# Autodesk Inventor assembly: Custom Cover Assembly
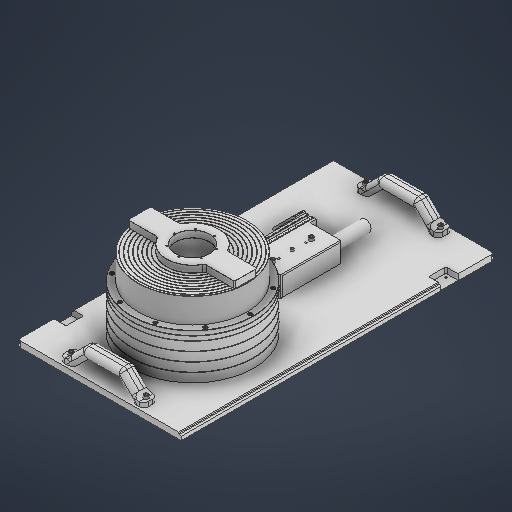
[picture p0: Inventor's stored thumbnail of the model, 512x512]
Saved by Autodesk Inventor 2025 (Build 290162000, 162)
## iProperties
Created: 2024-04-26
Part Number: Custom Cover Assembly
Document SubType Name: Assembly
Designer: Thienan Hoang
Author: Thienan Hoang
## Documents named in this file (23)
- C:\Users\mayhe\OneDrive\Documents\GitHub\In-situ-monitoring-of-powder-bed-fusion-additive-manufacturing\system_development\custom-cover\v0.1\hardware design\Custom Cover Full Assembly.iam
- C:\Users\mayhe\OneDrive\Documents\GitHub\In-situ-monitoring-of-powder-bed-fusion-additive-manufacturing\system_development\custom-cover\v0.1\hardware design\cover\Updated Cover.ipt
- C:\Users\mayhe\OneDrive\Documents\GitHub\In-situ-monitoring-of-powder-bed-fusion-additive-manufacturing\system_development\laser-vibrometer\v0.1\Hardware_design\Updated Laser Scanner.ipt
- C:\Users\mayhe\OneDrive\Documents\GitHub\In-situ-monitoring-of-powder-bed-fusion-additive-manufacturing\system_development\laser-vibrometer\v0.1\Hardware_design\Updated Laser Bracket.ipt
- C:\Users\mayhe\OneDrive\Documents\GitHub\In-situ-monitoring-of-powder-bed-fusion-additive-manufacturing\system_development\custom-cover\v0.1\hardware design\fasteners-standoffs\25-4136.ipt
- C:\Users\mayhe\OneDrive\Documents\GitHub\In-situ-monitoring-of-powder-bed-fusion-additive-manufacturing\system_development\custom-cover\v0.1\hardware design\fasteners-standoffs\11-4310.ipt
- C:\Users\mayhe\OneDrive\Documents\GitHub\In-situ-monitoring-of-powder-bed-fusion-additive-manufacturing\system_development\custom-cover\v0.1\hardware design\8020-parts\20-2020-160-CL.ipt
- C:\Users\mayhe\OneDrive\Documents\GitHub\In-situ-monitoring-of-powder-bed-fusion-additive-manufacturing\system_development\custom-cover\v0.1\hardware design\8020-parts\14159_m.ipt
- C:\Users\mayhe\OneDrive\Documents\GitHub\In-situ-monitoring-of-powder-bed-fusion-additive-manufacturing\system_development\galvo-scanner\V0.1\hardware design\GVS102.iam
- C:\Users\mayhe\OneDrive\Documents\GitHub\In-situ-monitoring-of-powder-bed-fusion-additive-manufacturing\system_development\custom-cover\v0.1\hardware design\8020-parts\20-2020-200-CL.ipt
- C:\Users\mayhe\OneDrive\Documents\GitHub\In-situ-monitoring-of-powder-bed-fusion-additive-manufacturing\system_development\custom-cover\v0.1\hardware design\8020-parts\25-1964.ipt
- C:\Users\mayhe\OneDrive\Documents\GitHub\In-situ-monitoring-of-powder-bed-fusion-additive-manufacturing\system_development\custom-cover\v0.1\hardware design\cylinder-parts\whole-pieces\Cylinder Spacer Bottom.ipt
- C:\Users\mayhe\OneDrive\Documents\GitHub\In-situ-monitoring-of-powder-bed-fusion-additive-manufacturing\system_development\custom-cover\v0.1\hardware design\cylinder-parts\whole-pieces\Cylinder Spacer Top.ipt
- C:\Users\mayhe\OneDrive\Documents\GitHub\In-situ-monitoring-of-powder-bed-fusion-additive-manufacturing\system_development\custom-cover\v0.1\hardware design\cylinder-parts\whole-pieces\Cylinder Slidey Bit.iam
- C:\Users\mayhe\OneDrive\Documents\GitHub\In-situ-monitoring-of-powder-bed-fusion-additive-manufacturing\system_development\custom-cover\v0.1\hardware design\cylinder-parts\whole-pieces\Cylinder Spacer 25mm.ipt
- C:\Users\mayhe\OneDrive\Documents\GitHub\In-situ-monitoring-of-powder-bed-fusion-additive-manufacturing\system_development\custom-cover\v0.1\hardware design\cylinder-parts\whole-pieces\Head Thing.ipt
- C:\Users\mayhe\OneDrive\Documents\GitHub\In-situ-monitoring-of-powder-bed-fusion-additive-manufacturing\system_development\custom-cover\v0.1\hardware design\cylinder-parts\whole-pieces\Cylinder Bottom.ipt
- C:\Users\mayhe\OneDrive\Documents\GitHub\In-situ-monitoring-of-powder-bed-fusion-additive-manufacturing\system_development\custom-cover\v0.1\hardware design\cover\Handles.ipt
- C:\Users\mayhe\OneDrive\Documents\GitHub\In-situ-monitoring-of-powder-bed-fusion-additive-manufacturing\system_development\custom-cover\v0.1\hardware design\fasteners-standoffs\ANSI B18.3.1M - M2x0.4 x 20(1).ipt
- C:\Users\mayhe\OneDrive\Documents\GitHub\In-situ-monitoring-of-powder-bed-fusion-additive-manufacturing\system_development\custom-cover\v0.1\hardware design\fasteners-standoffs\ANSI B18.3.1M - M6x1 x 20(1).ipt
- C:\Users\mayhe\OneDrive\Documents\GitHub\In-situ-monitoring-of-powder-bed-fusion-additive-manufacturing\system_development\custom-cover\v0.1\hardware design\fasteners-standoffs\ANSI B18.3.1M - M6x1 x 10(1).ipt
- C:\Users\mayhe\OneDrive\Documents\GitHub\In-situ-monitoring-of-powder-bed-fusion-additive-manufacturing\system_development\custom-cover\v0.1\hardware design\fasteners-standoffs\ANSI B18.3.1M - M4x0.7 x 6(1).ipt
- C:\Users\mayhe\OneDrive\Documents\GitHub\In-situ-monitoring-of-powder-bed-fusion-additive-manufacturing\system_development\custom-cover\v0.1\hardware design\fasteners-standoffs\ANSI B18.3.1M - M5x0.8 x 100(1).ipt
## Components (58 placed, 22 different names)
1. Updated Cover:1 — Mate:15, Mate:17, Mate:18, Mate:19, Mate:20, Mate:32, Mate:33, Flush:5, Mate:48, Mate:82, Mate:86, Mate:98, Mate:106, Mate:107, Mate:108, Mate:109
2. 11-4310:10 — Mate:125
3. 11-4310:11 — Mate:126
4. 11-4310:12 — Mate:127
5. 11-4310:13 — Mate:128
6. GVS102:1 [sub-assembly] — Mate:66, Mate:67, Angle:2
7. 20-2020-200-CL:1 — Mate:69, Flush:8, Mate:85, Angle:2, Mate:122, Mate:123, Mate:124
8. 25-1964:1 — Mate:66, Mate:67, Mate:69, Flush:8, Mate:85
9. Updated Laser Bracket:1 — Flush:9, Mate:83, Rotational:15, Mate:86, Insert:22, Insert:23, Insert:24, Mate:125, Mate:126, Mate:127, Mate:128
10. Updated Laser Scanner:1 — Rotational:15
11. Head Thing:1 — Mate:110, Mate:111, Insert:11, Insert:12, Insert:13, Insert:14, Insert:15, Insert:16, Insert:17
12. Cylinder Bottom:1 — Mate:98, Mate:99, Mate:100
13. Cylinder Spacer Bottom:1 — Mate:99, Mate:100, Mate:101, Mate:102, Mate:122, Mate:123, Mate:124
14. Cylinder Spacer Top:1 — Mate:101, Mate:102, Mate:103, Mate:104
15. Cylinder Spacer 25mm:1 — Mate:103, Mate:104, Mate:105, Rotational:16
16. Cylinder Slidey Bit:1 [sub-assembly] — Mate:105, Rotational:16, Mate:110, Mate:111, Mate:112, Mate:113, Mate:114, Mate:115, Mate:116, Mate:117, Mate:118, Mate:119, Mate:120, Mate:121
17. Handles:1 — Mate:108, Mate:109, Insert:18, Insert:19
18. Handles:2 — Mate:106, Mate:107, Insert:20, Insert:21
19. 25-4136:1 — Mate:5, Mate:6, Mate:9, Mate:10, Flush:1, Flush:2, Mate:15, Mate:17, Mate:18, Rotational:2, Rigid:1
20. 20-2020-160-CL:1 — Flush:1, Mate:11, Mate:12, Flush:9, Mate:83
21. 11-4310:1 — Mate:5, Mate:8
22. 11-4310:2 — Mate:6, Mate:7
23. 14159_m:1 — Mate:8, Mate:10, Mate:13, Mate:14
24. 14159_m:2 — Mate:7, Mate:9, Mate:11, Mate:12
25. 20-2020-160-CL:2 — Flush:2, Mate:13, Mate:14, Mate:56
26. 11-4310:3 — Rotational:2
27. 11-4310:4 — Rigid:1
28. 25-4136:3 — Mate:19, Mate:20, Rotational:3, Rotational:4, Rotational:5, Rotational:6, Mate:23, Mate:32, Mate:33, Mate:82
29. 11-4310:6 — Rotational:3
30. 11-4310:7 — Rotational:4
31. 11-4310:8 — Rotational:5, Mate:21
32. 11-4310:9 — Rotational:6, Mate:22
33. 14159_m:3 — Mate:22, Mate:56
34. 14159_m:4 — Mate:21, Mate:23
35. Forged Socket Head Cap Screw - Metric M2x0.4 x 20:1 — Insert:11
36. Forged Socket Head Cap Screw - Metric M2x0.4 x 20:2 — Insert:12
37. Forged Socket Head Cap Screw - Metric M2x0.4 x 20:3 — Insert:13
38. Forged Socket Head Cap Screw - Metric M2x0.4 x 20:4 — Insert:14
39. Forged Socket Head Cap Screw - Metric M2x0.4 x 20:5 — Insert:15
40. Forged Socket Head Cap Screw - Metric M2x0.4 x 20:6 — Insert:16
41. Forged Socket Head Cap Screw - Metric M2x0.4 x 20:7 — Insert:17
42. Forged Socket Head Cap Screw - Metric M6x1 x 20:1 — Insert:18
43. Forged Socket Head Cap Screw - Metric M6x1 x 20:2 — Insert:19
44. Forged Socket Head Cap Screw - Metric M6x1 x 20:3 — Insert:20
45. Forged Socket Head Cap Screw - Metric M6x1 x 20:4 — Insert:21
46. Forged Socket Head Cap Screw - Metric M6x1 x 10:1 — Insert:22
47. Forged Socket Head Cap Screw - Metric M6x1 x 10:2 — Insert:23
48. Forged Socket Head Cap Screw - Metric M4x0.7 x 6:1 — Insert:24
49. Forged Socket Head Cap Screw - Metric M5x0.8 x 100:1 — Mate:112
50. Forged Socket Head Cap Screw - Metric M5x0.8 x 100:3 — Mate:118
51. Forged Socket Head Cap Screw - Metric M5x0.8 x 100:4 — Mate:115
52. Forged Socket Head Cap Screw - Metric M5x0.8 x 100:5 — Mate:113
53. Forged Socket Head Cap Screw - Metric M5x0.8 x 100:6 — Mate:120
54. Forged Socket Head Cap Screw - Metric M5x0.8 x 100:7 — Mate:121
55. Forged Socket Head Cap Screw - Metric M5x0.8 x 100:8 — Mate:119
56. Forged Socket Head Cap Screw - Metric M5x0.8 x 100:9 — Mate:117
57. Forged Socket Head Cap Screw - Metric M5x0.8 x 100:10 — Mate:116
58. Forged Socket Head Cap Screw - Metric M5x0.8 x 100:11 — Mate:114
## Relationships (89: Mate 60, Insert 14, RevoluteJoint 7, Flush 6, WeldJoint 1, Angle 1)
- Mate:5: 25-4136:1 ↔ 11-4310:1
- Mate:6: 25-4136:1 ↔ 11-4310:2
- Mate:7: 11-4310:2 ↔ 14159_m:2
- Mate:8: 11-4310:1 ↔ 14159_m:1
- Mate:9 (1.5 mm): 25-4136:1 ↔ 14159_m:2
- Mate:10 (1.5 mm): 25-4136:1 ↔ 14159_m:1
- Flush:1: 25-4136:1 ↔ 20-2020-160-CL:1
- Flush:2: 25-4136:1 ↔ 20-2020-160-CL:2
- Mate:11: 20-2020-160-CL:1 ↔ 14159_m:2
- Mate:12 (1.5 mm): 20-2020-160-CL:1 ↔ 14159_m:2
- Mate:13: 14159_m:1 ↔ 20-2020-160-CL:2
- Mate:14 (1.45 mm): 14159_m:1 ↔ 20-2020-160-CL:2
- Mate:15: Updated Cover:1 ↔ 25-4136:1
- Mate:17: Updated Cover:1 ↔ 25-4136:1
- Mate:18: Updated Cover:1 ↔ 25-4136:1
- Rotational:2 [RevoluteJoint]: 25-4136:1 ↔ 11-4310:3
- Rigid:1 [WeldJoint]: 25-4136:1 ↔ 11-4310:4
- Mate:19: Updated Cover:1 ↔ 25-4136:3
- Mate:20: Updated Cover:1 ↔ 25-4136:3
- Rotational:3 [RevoluteJoint]: 25-4136:3 ↔ 11-4310:6
- Rotational:4 [RevoluteJoint]: 25-4136:3 ↔ 11-4310:7
- Rotational:5 [RevoluteJoint]: 25-4136:3 ↔ 11-4310:8
- Rotational:6 [RevoluteJoint]: 25-4136:3 ↔ 11-4310:9
- Mate:21: 11-4310:8 ↔ 14159_m:4
- Mate:22: 11-4310:9 ↔ 14159_m:3
- Mate:23 (1.5 mm): 25-4136:3 ↔ 14159_m:4
- Mate:32: Updated Cover:1 ↔ 25-4136:3
- Mate:33: Updated Cover:1 ↔ 25-4136:3
- Flush:5 (180 mm): Updated Cover:1
- Mate:48: Updated Cover:1
- Flush:6 (38 mm)
- Mate:56: 20-2020-160-CL:2 ↔ 14159_m:3
- Mate:66: GVS102:1 ↔ 25-1964:1
- Mate:67 (1.5 mm): GVS102:1 ↔ 25-1964:1
- Mate:69 (0.52 mm): 20-2020-200-CL:1 ↔ 25-1964:1
- Flush:8 (34 mm): 20-2020-200-CL:1 ↔ 25-1964:1
- Mate:82: Updated Cover:1 ↔ 25-4136:3
- Flush:9: Updated Laser Bracket:1 ↔ 20-2020-160-CL:1
- Mate:83: Updated Laser Bracket:1 ↔ 20-2020-160-CL:1
- Mate:85: 20-2020-200-CL:1 ↔ 25-1964:1
- Rotational:15 [RevoluteJoint]: Updated Laser Bracket:1 ↔ Updated Laser Scanner:1
- Mate:86 (1.5 mm): Updated Cover:1 ↔ Updated Laser Bracket:1
- Angle:2 (0 deg): GVS102:1 ↔ 20-2020-200-CL:1
- Mate:98: Updated Cover:1 ↔ Cylinder Bottom:1
- Mate:99: Cylinder Bottom:1 ↔ Cylinder Spacer Bottom:1
- Mate:100: Cylinder Bottom:1 ↔ Cylinder Spacer Bottom:1
- Mate:101: Cylinder Spacer Bottom:1 ↔ Cylinder Spacer Top:1
- Mate:102: Cylinder Spacer Bottom:1 ↔ Cylinder Spacer Top:1
- Mate:103: Cylinder Spacer Top:1 ↔ Cylinder Spacer 25mm:1
- Mate:104: Cylinder Spacer Top:1 ↔ Cylinder Spacer 25mm:1
- Mate:105: Cylinder Spacer 25mm:1 ↔ Cylinder Slidey Bit:1
- Rotational:16 [RevoluteJoint]: Cylinder Spacer 25mm:1 ↔ Cylinder Slidey Bit:1
- Mate:106: Updated Cover:1 ↔ Handles:2
- Mate:107: Updated Cover:1 ↔ Handles:2
- Mate:108: Updated Cover:1 ↔ Handles:1
- Mate:109: Updated Cover:1 ↔ Handles:1
- Mate:110: Head Thing:1 ↔ Cylinder Slidey Bit:1
- Mate:111: Head Thing:1 ↔ Cylinder Slidey Bit:1
- Insert:11: Head Thing:1 ↔ Forged Socket Head Cap Screw - Metric M2x0.4 x 20:1
- Insert:12: Head Thing:1 ↔ Forged Socket Head Cap Screw - Metric M2x0.4 x 20:2
- Insert:13: Head Thing:1 ↔ Forged Socket Head Cap Screw - Metric M2x0.4 x 20:3
- Insert:14: Head Thing:1 ↔ Forged Socket Head Cap Screw - Metric M2x0.4 x 20:4
- Insert:15: Head Thing:1 ↔ Forged Socket Head Cap Screw - Metric M2x0.4 x 20:5
- Insert:16: Head Thing:1 ↔ Forged Socket Head Cap Screw - Metric M2x0.4 x 20:6
- Insert:17: Head Thing:1 ↔ Forged Socket Head Cap Screw - Metric M2x0.4 x 20:7
- Insert:18: Handles:1 ↔ Forged Socket Head Cap Screw - Metric M6x1 x 20:1
- Insert:19: Handles:1 ↔ Forged Socket Head Cap Screw - Metric M6x1 x 20:2
- Insert:20: Handles:2 ↔ Forged Socket Head Cap Screw - Metric M6x1 x 20:3
- Insert:21: Handles:2 ↔ Forged Socket Head Cap Screw - Metric M6x1 x 20:4
- Insert:22: Updated Laser Bracket:1 ↔ Forged Socket Head Cap Screw - Metric M6x1 x 10:1
- Insert:23: Updated Laser Bracket:1 ↔ Forged Socket Head Cap Screw - Metric M6x1 x 10:2
- Insert:24: Updated Laser Bracket:1 ↔ Forged Socket Head Cap Screw - Metric M4x0.7 x 6:1
- Mate:112: Cylinder Slidey Bit:1 ↔ Forged Socket Head Cap Screw - Metric M5x0.8 x 100:1
- Mate:113: Cylinder Slidey Bit:1 ↔ Forged Socket Head Cap Screw - Metric M5x0.8 x 100:5
- Mate:114: Cylinder Slidey Bit:1 ↔ Forged Socket Head Cap Screw - Metric M5x0.8 x 100:11
- Mate:115: Cylinder Slidey Bit:1 ↔ Forged Socket Head Cap Screw - Metric M5x0.8 x 100:4
- Mate:116: Cylinder Slidey Bit:1 ↔ Forged Socket Head Cap Screw - Metric M5x0.8 x 100:10
- Mate:117: Cylinder Slidey Bit:1 ↔ Forged Socket Head Cap Screw - Metric M5x0.8 x 100:9
- Mate:118: Cylinder Slidey Bit:1 ↔ Forged Socket Head Cap Screw - Metric M5x0.8 x 100:3
- Mate:119: Cylinder Slidey Bit:1 ↔ Forged Socket Head Cap Screw - Metric M5x0.8 x 100:8
- Mate:120: Cylinder Slidey Bit:1 ↔ Forged Socket Head Cap Screw - Metric M5x0.8 x 100:6
- Mate:121: Cylinder Slidey Bit:1 ↔ Forged Socket Head Cap Screw - Metric M5x0.8 x 100:7
- Mate:122: 20-2020-200-CL:1 ↔ Cylinder Spacer Bottom:1
- Mate:123: 20-2020-200-CL:1 ↔ Cylinder Spacer Bottom:1
- Mate:124: 20-2020-200-CL:1 ↔ Cylinder Spacer Bottom:1
- Mate:125: 11-4310:10 ↔ Updated Laser Bracket:1
- Mate:126: 11-4310:11 ↔ Updated Laser Bracket:1
- Mate:127: 11-4310:12 ↔ Updated Laser Bracket:1
- Mate:128: 11-4310:13 ↔ Updated Laser Bracket:1
